# Autodesk Inventor assembly: X_Carriage_V2_0
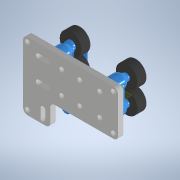
[picture p0: Inventor's stored thumbnail of the model, 180x180]
Saved by Autodesk Inventor 2021 (Build 250183000, 183)
## iProperties
Created: 2021-06-13
Part Number: X_Carriage_V2_0
Document SubType Name: Assembly
Designer: Jorian Brusind
Author: Jorian Brusind
## Documents named in this file (6)
- C:\Users\Jorian Brusind\Documents\GitHub\PersonalProjects\HyperRail\Inventor Files\X_Carriage_V2_0.iam
- C:\Users\Jorian Brusind\Documents\GitHub\PersonalProjects\HyperRail\Inventor Files\X_Carriage_Plate.ipt
- C:\Users\Jorian Brusind\Documents\GitHub\PersonalProjects\HyperRail\Inventor Files\11mm_BearingWheel.ipt
- C:\Users\Jorian Brusind\Documents\GitHub\PersonalProjects\HyperRail\Inventor Files\Belt_Restraint.ipt
- C:\Users\Jorian Brusind\Documents\GitHub\PersonalProjects\HyperRail\Inventor Files\4mm_Roller_Spacer_simple.ipt
- C:\Users\Jorian Brusind\Documents\GitHub\PersonalProjects\HyperRail\Inventor Files\4mm_Roller_Spacer_simple3mm.ipt
## Components (10 placed, 5 different names)
1. X_Carriage_Plate:1 — Mate:1, Mate:2, Mate:3, Mate:5, Mate:7, Mate:8, Mate:9, Mate:10, Mate:12, Mate:13, Mate:14, Mate:24, Mate:25, Mate:26
2. 11mm_BearingWheel:1 — Mate:1, Mate:6, Flush:2
3. 11mm_BearingWheel:2 — Mate:5, Mate:6, Flush:1
4. 11mm_BearingWheel:3 — Mate:3, Mate:4, Flush:1, Flush:3, Mate:29, Mate:30, Mate:31
5. 11mm_BearingWheel:4 — Mate:2, Mate:4, Flush:2, Flush:3, Mate:7
6. 11mm_BearingWheel:5 — Mate:8, Mate:9, Mate:10
7. Belt_Restraint:1 — Angle:1, Mate:28, Mate:29, Angle:2
8. 4mm_Roller_Spacer_simple:2 — Mate:12, Mate:13, Mate:14, Angle:1, Mate:28
9. Belt_Restraint:2 — Mate:30, Mate:31, Angle:2
10. 4mm_Roller_Spacer_simple3mm:1 — Mate:24, Mate:25, Mate:26
## Relationships (25: Mate 20, Flush 3, Angle 2)
- Mate:1: X_Carriage_Plate:1 ↔ 11mm_BearingWheel:1
- Mate:2: X_Carriage_Plate:1 ↔ 11mm_BearingWheel:4
- Mate:3 (2.75 mm): X_Carriage_Plate:1 ↔ 11mm_BearingWheel:3
- Mate:4 (62 mm): 11mm_BearingWheel:3 ↔ 11mm_BearingWheel:4
- Mate:5 (2.75 mm): X_Carriage_Plate:1 ↔ 11mm_BearingWheel:2
- Mate:6 (62 mm): 11mm_BearingWheel:1 ↔ 11mm_BearingWheel:2
- Flush:1: 11mm_BearingWheel:2 ↔ 11mm_BearingWheel:3
- Flush:2: 11mm_BearingWheel:1 ↔ 11mm_BearingWheel:4
- Flush:3: 11mm_BearingWheel:3 ↔ 11mm_BearingWheel:4
- Mate:7 (23 mm): X_Carriage_Plate:1 ↔ 11mm_BearingWheel:4
- Mate:8 (2.75 mm): X_Carriage_Plate:1 ↔ 11mm_BearingWheel:5
- Mate:9 (-10 mm): X_Carriage_Plate:1 ↔ 11mm_BearingWheel:5
- Mate:10 (23 mm): X_Carriage_Plate:1 ↔ 11mm_BearingWheel:5
- Mate:12: X_Carriage_Plate:1 ↔ 4mm_Roller_Spacer_simple:2
- Mate:13: X_Carriage_Plate:1 ↔ 4mm_Roller_Spacer_simple:2
- Mate:14: X_Carriage_Plate:1 ↔ 4mm_Roller_Spacer_simple:2
- Mate:24: X_Carriage_Plate:1 ↔ 4mm_Roller_Spacer_simple3mm:1
- Mate:25: X_Carriage_Plate:1 ↔ 4mm_Roller_Spacer_simple3mm:1
- Mate:26: X_Carriage_Plate:1 ↔ 4mm_Roller_Spacer_simple3mm:1
- Angle:1 (0 deg): Belt_Restraint:1 ↔ 4mm_Roller_Spacer_simple:2
- Mate:28: Belt_Restraint:1 ↔ 4mm_Roller_Spacer_simple:2
- Mate:29: 11mm_BearingWheel:3 ↔ Belt_Restraint:1
- Mate:30: 11mm_BearingWheel:3 ↔ Belt_Restraint:2
- Mate:31: 11mm_BearingWheel:3 ↔ Belt_Restraint:2
- Angle:2 (0 deg): Belt_Restraint:1 ↔ Belt_Restraint:2
